# Autodesk Inventor assembly: AMESLaunching
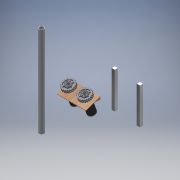
[picture p0: Inventor's stored thumbnail of the model, 180x180]
Saved by Autodesk Inventor 2017 (Build 210142000, 142)
## iProperties
Created: 2017-11-02
Part Number: AMESLaunching
Document SubType Name: Assembly
Designer: Aidan_Moga
Author: Aidan_Moga
## Documents named in this file (8)
- C:\Users\Aidan_Moga\Documents\Robotics\AMESLauncher\AMESLaunching.iam
- C:\Users\Aidan_Moga\Documents\Robotics\AMESLauncher\Beam_Supports.ipt
- C:\Users\Aidan_Moga\Documents\Robotics\AMESLauncher\70DegreeWoodHinge.ipt
- C:\Users\Aidan_Moga\Documents\Robotics\SIM_Motor.ipt
- C:\Users\Aidan_Moga\Documents\Robotics\am-0320a_8mm_Key_Hub.ipt
- C:\Users\Aidan_Moga\Documents\Robotics\AMESLauncher\Motor_Plate.ipt
- C:\Users\Aidan_Moga\Documents\Robotics\AMESLauncher\4 in HiGrip Wheel.iam
- C:\Users\Aidan_Moga\Documents\Robotics\AMESLauncher\Barrel.ipt
## Components (12 placed, 7 different names)
1. Beam_Supports:1 — Mate:1
2. Beam_Supports:2 — Mate:1, Mate:2
3. 70DegreeWoodHinge:1 — Mate:2, Rigid:2
4. 70DegreeWoodHinge:2 — Rigid:1
5. SIM_Motor:1 — Cylindrical:1, Mate:3, Angle:1, Angle:4, Mate:10
6. am-0320a_8mm_Key_Hub:1 — Cylindrical:1, Mate:3, Mate:4, Mate:5
7. Motor_Plate:1 — Angle:3, Angle:4, Mate:9, Mate:10, Rigid:1, Rigid:2
8. 4 in HiGrip Wheel:1 [sub-assembly] — Angle:1, Mate:4, Mate:5
9. SIM_Motor:2 — Angle:3, Mate:9
10. am-0320a_8mm_Key_Hub:2
11. 4 in HiGrip Wheel:2 [sub-assembly]
12. Barrel:1
## Relationships (18: Mate 10, Angle 4, CylindricalJoint 2, WeldJoint 2)
- Mate:1 (190.5 mm): Beam_Supports:1 ↔ Beam_Supports:2
- Mate:2: Beam_Supports:2 ↔ 70DegreeWoodHinge:1
- Cylindrical:1: SIM_Motor:1 ↔ am-0320a_8mm_Key_Hub:1
- Mate:3: SIM_Motor:1 ↔ am-0320a_8mm_Key_Hub:1
- Angle:1 (180 deg): SIM_Motor:1 ↔ 4 in HiGrip Wheel:1
- Mate:4: am-0320a_8mm_Key_Hub:1 ↔ 4 in HiGrip Wheel:1
- Mate:5: am-0320a_8mm_Key_Hub:1 ↔ 4 in HiGrip Wheel:1
- [CylindricalJoint]: SIM_Motor:2 ↔ am-0320a_8mm_Key_Hub:2
- [Mate]: SIM_Motor:2 ↔ am-0320a_8mm_Key_Hub:2
- [Angle] (180 deg): SIM_Motor:2 ↔ 4 in HiGrip Wheel:2
- [Mate]: am-0320a_8mm_Key_Hub:2 ↔ 4 in HiGrip Wheel:2
- [Mate]: am-0320a_8mm_Key_Hub:2 ↔ 4 in HiGrip Wheel:2
- Angle:3 (0 deg): Motor_Plate:1 ↔ SIM_Motor:2
- Angle:4 (0 deg): SIM_Motor:1 ↔ Motor_Plate:1
- Mate:9: Motor_Plate:1 ↔ SIM_Motor:2
- Mate:10: SIM_Motor:1 ↔ Motor_Plate:1
- Rigid:1 [WeldJoint]: 70DegreeWoodHinge:2 ↔ Motor_Plate:1
- Rigid:2 [WeldJoint]: 70DegreeWoodHinge:1 ↔ Motor_Plate:1
## Named parameters: d8_d4 = 0 mm, d9_d5 = 180 deg, d10_d6 = 0 mm, d11_d7 = 0 mm, d12_d2 = -30.001536 deg, d13_d3 = -0.254 mm
